# Autodesk Inventor assembly: ELEV_000_FULLASMBLY
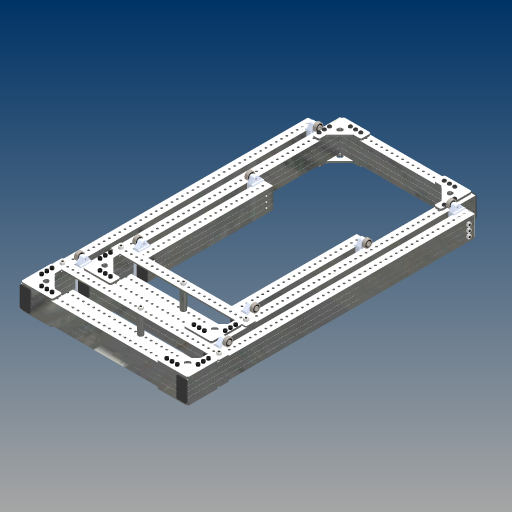
[picture p0: Inventor's stored thumbnail of the model, 512x512]
Saved by Autodesk Inventor 2024.3 (Build 283343000, 343)
## iProperties
Created: 2024-11-25
Part Number: ELEV_000_FULLASMBLY
Document SubType Name: Assembly
Designer: Kenji
Mass: 3407.89 g
Surface Area: 12378 cm^2
Volume: 1206.36 cm^3
Density: 2.82493 g/cm^3
Author: Kenji
## Documents named in this file (30)
- C:\Users\Kenji\Documents\GitHub\1622-2024-Casino-Clash-CAD-A-Thon\Elevator\ELEV_000_FULLASMBLY.iam
- C:\Users\Kenji\Documents\GitHub\1622-2024-Casino-Clash-CAD-A-Thon\Elevator\ELEV_001_BAR1(27.500 in).ipt
- C:\Users\Kenji\Documents\GitHub\1622-2024-Casino-Clash-CAD-A-Thon\Elevator\ELEV_002_BAR2(14.000 in).ipt
- C:\Users\Kenji\Documents\GitHub\1622-2024-Casino-Clash-CAD-A-Thon\Elevator\ELEV_003_BAR3(25.000 in).ipt
- C:\Users\Kenji\Documents\GitHub\1622-2024-Casino-Clash-CAD-A-Thon\COTS Library\Motion\BearingBlocks\ElevatorBlocks\WCP-0897_InlineBearingBlock.iam
- C:\Users\Kenji\Documents\GitHub\1622-2024-Casino-Clash-CAD-A-Thon\Elevator\ELEV_004_BAR4(12.000 in).ipt
- C:\Users\Kenji\Documents\GitHub\1622-2024-Casino-Clash-CAD-A-Thon\Elevator\ELEV_005_SUPBRK1.ipt
- C:\Users\Kenji\Documents\GitHub\1622-2024-Casino-Clash-CAD-A-Thon\COTS Library\Fasteners\Nuts\COTS_90633A411_Low-Strength Steel Thin Nylon-Insert Locknut_10-32.ipt
- C:\Users\Kenji\Documents\GitHub\1622-2024-Casino-Clash-CAD-A-Thon\Elevator\ELEV_006_SUPBRK1_THRD.ipt
- C:\Users\Kenji\Documents\GitHub\1622-2024-Casino-Clash-CAD-A-Thon\COTS Library\Fasteners\Bolts\Socket-Head\10-32\COTS_90044A121_Black-Oxide Alloy Steel Socket Head Screw_10-32_2.5in.ipt
- C:\Users\Kenji\Documents\GitHub\1622-2024-Casino-Clash-CAD-A-Thon\COTS Library\Fasteners\Bolts\Socket-Head\10-32\COTS_90044A202_Black-Oxide Alloy Steel Socket Head Screw_1-.375.ipt
- C:\Users\Kenji\Documents\GitHub\1622-2024-Casino-Clash-CAD-A-Thon\COTS Library\Fasteners\Bolts\Socket-Head\10-32\COTS_91251A342_Black-Oxide Alloy Steel Socket Head Screw_.5in.ipt
- C:\Users\Kenji\Documents\GitHub\1622-2024-Casino-Clash-CAD-A-Thon\Elevator\ELEV_007_SUPBRK2.ipt
- C:\Users\Kenji\Documents\GitHub\1622-2024-Casino-Clash-CAD-A-Thon\COTS Library\Fasteners\Bolts\Socket-Head\10-32\COTS_91251A359_Black-Oxide Alloy Steel Socket Head Screw_10-32_2_3-4in.ipt
- C:\Users\Kenji\Documents\GitHub\1622-2024-Casino-Clash-CAD-A-Thon\COTS Library\Fasteners\Nuts\COTS_90631A411_Low-Strength Steel Nylon-Insert Locknut_10-32.ipt
- C:\Users\Kenji\Documents\GitHub\1622-2024-Casino-Clash-CAD-A-Thon\Elevator\ELEV_008_SUPBRK3.ipt
- C:\Users\Kenji\Documents\GitHub\1622-2024-Casino-Clash-CAD-A-Thon\Elevator\ELEV_010_BOLTCOVER2.ipt
- C:\Users\Kenji\Documents\GitHub\1622-2024-Casino-Clash-CAD-A-Thon\Elevator\ELEV_011_EXTRUENDCAP.ipt
- C:\Users\Kenji\Documents\GitHub\1622-2024-Casino-Clash-CAD-A-Thon\Elevator\ELEV_012_SUPBRK2_THRD.ipt
- C:\Users\Kenji\Documents\GitHub\1622-2024-Casino-Clash-CAD-A-Thon\Elevator\ELEV_013_BAR5(12.000 in).ipt
- C:\Users\Kenji\Documents\GitHub\1622-2024-Casino-Clash-CAD-A-Thon\Elevator\ELEV_015_CRSHBLCK1.ipt
- C:\Users\Kenji\Documents\GitHub\1622-2024-Casino-Clash-CAD-A-Thon\Elevator\ELEV_016_SUPBAR1.ipt
- C:\Users\Kenji\Documents\GitHub\1622-2024-Casino-Clash-CAD-A-Thon\Elevator\ELEV_017_SPACER1.ipt
- C:\Users\Kenji\Documents\GitHub\1622-2024-Casino-Clash-CAD-A-Thon\Elevator\ELEV_018_SUPBAR2.ipt
- C:\Users\Kenji\Documents\GitHub\1622-2024-Casino-Clash-CAD-A-Thon\Elevator\ELEV_000_FULLASMBLY\AIP\FEA\ew6g7bhkw.fins
- C:\Users\Kenji\Documents\GitHub\1622-2024-Casino-Clash-CAD-A-Thon\Elevator\ELEV_000_FULLASMBLY\AIP\FEA\ew6g7bhkw.fsat
- C:\Users\Kenji\Documents\GitHub\1622-2024-Casino-Clash-CAD-A-Thon\Elevator\ELEV_000_FULLASMBLY\AIP\FEA\ew6g7bhkw.ftes
- C:\Users\Kenji\Documents\GitHub\1622-2024-Casino-Clash-CAD-A-Thon\Elevator\ELEV_000_FULLASMBLY\AIP\FEA\ew6g7bhkw.fwiz
- C:\Users\Kenji\Documents\GitHub\1622-2024-Casino-Clash-CAD-A-Thon\Elevator\ELEV_000_FULLASMBLY\AIP\FEA\ew6g7biao.fmsh
- C:\Users\Kenji\Documents\GitHub\1622-2024-Casino-Clash-CAD-A-Thon\Elevator\ELEV_000_FULLASMBLY\AIP\FEA\ew6g7bibk.fres
## Components (192 placed, 23 different names)
1. ELEV_001_BAR1(27.500 in):1 — Flush:1, Flush:2, Mate:1, Mate:2, Flush:7, Tangent:2, Mate:10, Flush:11, Mate:11, Mate:78, Mate:133, Mate:136, Mate:137, Mate:201, Mate:202, Mate:203, Mate:284, Mate:285, Mate:286, Mate:290, Mate:293
2. ELEV_001_BAR1(27.500 in):2 — Flush:1, Flush:2, Mate:1, Flush:3, Flush:4, Mate:3, Angle:1, Mate:4, Flush:8, Angle:2, Mate:74, Mate:128, Mate:131, Mate:198, Mate:199, Mate:200, Mate:287, Mate:288, Mate:289, Mate:291, Mate:292, Mate:294, Mate:295
3. ELEV_002_BAR2(14.000 in):1 — Flush:3, Flush:4, Mate:2, Mate:127, Flush:24, Mate:132, Mate:134, Mate:135
4. ELEV_003_BAR3(25.000 in):1 — Flush:5, Flush:6, Flush:7, Mate:8, Flush:10, Mate:9, Mate:82, Mate:186, Mate:187, Mate:188, Mate:211, Mate:228, Tangent:3, Tangent:4, Angle:5, Angle:6, Mate:265, Mate:266, Mate:267, Mate:312, Mate:313, Mate:316
5. ELEV_003_BAR3(25.000 in):2 — Flush:5, Flush:6, Tangent:1, Angle:2, Mate:5, Angle:3, Mate:6, Flush:9, Mate:12, Flush:12, Flush:13, Mate:13, Flush:14, Mate:14, Mate:16, Mate:62, Mate:86, Mate:189, Mate:190, Mate:191, Mate:192, Mate:193, Mate:194, Mate:207, Mate:208, Tangent:5, Flush:33
6. WCP-0897_InlineBearingBlock:1 [sub-assembly] — Mate:5, Angle:3, Mate:6, Flush:9, Mate:83, Mate:84
7. WCP-0897_InlineBearingBlock:2 [sub-assembly] — Mate:3, Angle:1, Mate:4, Tangent:1, Flush:8, Mate:71, Mate:72
8. WCP-0897_InlineBearingBlock:3 [sub-assembly] — Mate:8, Flush:10, Mate:9, Tangent:2, Mate:79, Mate:80
9. WCP-0897_InlineBearingBlock:4 [sub-assembly] — Mate:10, Flush:11, Mate:11, Mate:75, Mate:76
10. ELEV_004_BAR4(12.000 in):1 — Mate:12, Flush:12, Flush:13, Mate:17, Mate:18, Mate:19, Angle:4, Mate:20, Mate:42, Mate:45, Mate:60, Flush:15, Mate:61, Angle:8
11. ELEV_004_BAR4(12.000 in):2 — Mate:13, Flush:14, Mate:14, Flush:26, Flush:27, Mate:214, Mate:227, Flush:28, Angle:7
12. ELEV_005_SUPBRK1:1 — Mate:16, Mate:17, Mate:18, Mate:67, Mate:68, Mate:69, Mate:70
13. ELEV_005_SUPBRK1:2 — Mate:19, Angle:4, Mate:20, Mate:63, Mate:64, Mate:65, Mate:66
14. ELEV_006_SUPBRK1_THRD:1 — Mate:42, Mate:61, Mate:62, Mate:247, Mate:248
15. ELEV_006_SUPBRK1_THRD:2 — Mate:45, Mate:60, Flush:15, Mate:241, Mate:242, Mate:243, Mate:244
16. ELEV_008_SUPBRK3:1 — Mate:127, Flush:24, Mate:128, Mate:129, Mate:130, Mate:138, Mate:139, Mate:144, Mate:145
17. ELEV_008_SUPBRK3:2 — Mate:129, Mate:130, Mate:131, Mate:148, Mate:149
18. ELEV_008_SUPBRK3:3 — Mate:132, Mate:133, Mate:134, Mate:151, Mate:153
19. ELEV_008_SUPBRK3:4 — Mate:135, Mate:136, Mate:137, Mate:140, Mate:141, Mate:142, Mate:143
20. ELEV_011_EXTRUENDCAP:1 — Mate:189, Mate:190, Mate:191
21. ELEV_011_EXTRUENDCAP:3 — Mate:186, Mate:187, Mate:188, Mate:339
22. ELEV_011_EXTRUENDCAP:5 — Mate:198, Mate:199, Mate:200
23. ELEV_011_EXTRUENDCAP:6 — Mate:201, Mate:202, Mate:203
24. ELEV_011_EXTRUENDCAP:7 — Mate:192, Mate:193, Mate:194
25. ELEV_007_SUPBRK2:1 — Flush:26, Mate:227, Mate:228, Mate:229, Mate:230, Mate:231, Mate:232, Mate:233
26. ELEV_007_SUPBRK2:2 — Flush:27, Mate:207, Mate:208, Mate:212, Mate:213, Mate:217, Mate:218, Mate:219, Mate:220
27. ELEV_012_SUPBRK2_THRD:1 — Mate:211, Mate:229, Flush:28, Mate:239, Mate:240
28. ELEV_012_SUPBRK2_THRD:2 — Mate:212, Mate:213, Mate:214, Mate:235, Mate:332
29. ELEV_013_BAR5(12.000 in):1 — Mate:257, Flush:29, Mate:258, Mate:259, Flush:30, Mate:260, Angle:5, Angle:6, Flush:34, Mate:277, Mate:283, Mate:333, Mate:334, Mate:335
30. ELEV_013_BAR5(12.000 in):2 — Mate:261, Flush:31, Mate:262, Mate:263, Flush:32, Mate:264, Angle:7, Flush:33, Flush:34, Mate:279, Mate:281, Mate:336, Mate:337, Mate:338
31. WCP-0897_InlineBearingBlock:5 [sub-assembly] — Mate:257, Flush:29, Mate:258, Tangent:3, Tangent:4, Mate:270, Mate:271
32. WCP-0897_InlineBearingBlock:6 [sub-assembly] — Mate:259, Flush:30, Mate:260, Mate:274, Mate:275
33. WCP-0897_InlineBearingBlock:7 [sub-assembly] — Mate:261, Flush:31, Mate:262, Tangent:5, Mate:272, Mate:273
34. WCP-0897_InlineBearingBlock:8 [sub-assembly] — Mate:263, Flush:32, Mate:264, Mate:268, Mate:269
35. ELEV_011_EXTRUENDCAP:8 — Mate:265, Mate:266, Mate:267
36. ELEV_015_CRSHBLCK1:1 — Mate:284, Mate:285, Mate:286
37. ELEV_015_CRSHBLCK1:2 — Mate:287, Mate:288, Mate:289
38. ELEV_016_SUPBAR1:1 — Mate:290, Mate:291, Mate:292, Mate:301, Mate:303, Mate:305, Mate:310
39. ELEV_016_SUPBAR1:2 — Mate:293, Mate:294, Mate:295, Mate:296, Mate:297, Mate:298, Mate:299, Mate:304, Mate:306, Mate:307, Mate:308, Mate:339
40. COTS_90044A121_Black-Oxide Alloy Steel Socket Head Screw_10-32_2.5in:27 — Mate:296, Mate:297, Mate:302
41. COTS_90044A121_Black-Oxide Alloy Steel Socket Head Screw_10-32_2.5in:28 — Mate:298, Mate:299, Mate:300
42. COTS_90631A411_Low-Strength Steel Nylon-Insert Locknut_10-32:25 — Mate:300, Mate:301
43. COTS_90631A411_Low-Strength Steel Nylon-Insert Locknut_10-32:26 — Mate:302, Mate:303
44. ELEV_017_SPACER1:1 — Mate:304, Mate:305, Mate:306
45. COTS_90044A121_Black-Oxide Alloy Steel Socket Head Screw_10-32_2.5in:29 — Mate:307, Mate:308, Mate:309
46. COTS_90631A411_Low-Strength Steel Nylon-Insert Locknut_10-32:27 — Mate:309, Mate:310
47. ELEV_018_SUPBAR2:1 — Mate:312, Mate:313, Angle:8, Mate:314, Mate:315, Mate:317, Mate:318, Mate:319, Mate:320, Mate:325, Mate:326, Mate:327, Mate:328, Mate:340
48. ELEV_018_SUPBAR2:2 — Mate:314, Mate:315, Mate:316, Mate:323, Mate:324, Mate:330
49. COTS_90044A121_Black-Oxide Alloy Steel Socket Head Screw_10-32_2.5in:30 — Mate:318, Mate:319, Mate:321
50. COTS_90044A121_Black-Oxide Alloy Steel Socket Head Screw_10-32_2.5in:31 — Mate:317, Mate:320, Mate:322
51. COTS_90044A121_Black-Oxide Alloy Steel Socket Head Screw_10-32_2.5in:32 — Mate:327, Mate:328, Mate:329
52. COTS_90631A411_Low-Strength Steel Nylon-Insert Locknut_10-32:28 — Mate:322, Mate:323
53. COTS_90631A411_Low-Strength Steel Nylon-Insert Locknut_10-32:29 — Mate:321, Mate:324
54. ELEV_017_SPACER1:2 — Mate:325, Mate:326
55. COTS_90631A411_Low-Strength Steel Nylon-Insert Locknut_10-32:30 — Mate:329, Mate:330
56. ELEV_011_EXTRUENDCAP:9 — Mate:333, Mate:334, Mate:335, Mate:340
57. ELEV_011_EXTRUENDCAP:10 — Mate:336, Mate:337, Mate:338
58. COTS_90044A121_Black-Oxide Alloy Steel Socket Head Screw_10-32_2.5in:1 — Mate:63, Mate:64
59. COTS_90044A121_Black-Oxide Alloy Steel Socket Head Screw_10-32_2.5in:5
60. COTS_90044A121_Black-Oxide Alloy Steel Socket Head Screw_10-32_2.5in:6
61. COTS_90044A121_Black-Oxide Alloy Steel Socket Head Screw_10-32_2.5in:4 — Mate:65, Mate:66
62. COTS_90044A121_Black-Oxide Alloy Steel Socket Head Screw_10-32_2.5in:7
63. COTS_90044A121_Black-Oxide Alloy Steel Socket Head Screw_10-32_2.5in:8
64. COTS_90044A121_Black-Oxide Alloy Steel Socket Head Screw_10-32_2.5in:2 — Mate:67, Mate:69, Mate:245
65. COTS_90044A121_Black-Oxide Alloy Steel Socket Head Screw_10-32_2.5in:11
66. COTS_90044A121_Black-Oxide Alloy Steel Socket Head Screw_10-32_2.5in:12
67. COTS_90044A202_Black-Oxide Alloy Steel Socket Head Screw_1-.375:1 — Mate:71, Mate:72, Mate:73
68. COTS_90633A411_Low-Strength Steel Thin Nylon-Insert Locknut_10-32:1 — Mate:73, Mate:74
69. COTS_90044A202_Black-Oxide Alloy Steel Socket Head Screw_1-.375:2
70. COTS_90633A411_Low-Strength Steel Thin Nylon-Insert Locknut_10-32:2
71. COTS_90044A202_Black-Oxide Alloy Steel Socket Head Screw_1-.375:3
72. COTS_90633A411_Low-Strength Steel Thin Nylon-Insert Locknut_10-32:3
73. COTS_90633A411_Low-Strength Steel Thin Nylon-Insert Locknut_10-32:4 — Mate:77, Mate:78
74. COTS_90044A202_Black-Oxide Alloy Steel Socket Head Screw_1-.375:4 — Mate:75, Mate:76, Mate:77
75. COTS_90633A411_Low-Strength Steel Thin Nylon-Insert Locknut_10-32:5
76. COTS_90044A202_Black-Oxide Alloy Steel Socket Head Screw_1-.375:5
77. COTS_90633A411_Low-Strength Steel Thin Nylon-Insert Locknut_10-32:6
78. COTS_90044A202_Black-Oxide Alloy Steel Socket Head Screw_1-.375:6
79. COTS_91251A342_Black-Oxide Alloy Steel Socket Head Screw_.5in:1 — Mate:79, Mate:80, Mate:81
80. COTS_90633A411_Low-Strength Steel Thin Nylon-Insert Locknut_10-32:7 — Mate:81, Mate:82
81. COTS_91251A342_Black-Oxide Alloy Steel Socket Head Screw_.5in:2
82. COTS_90633A411_Low-Strength Steel Thin Nylon-Insert Locknut_10-32:8
83. COTS_91251A342_Black-Oxide Alloy Steel Socket Head Screw_.5in:3
84. COTS_90633A411_Low-Strength Steel Thin Nylon-Insert Locknut_10-32:9
85. COTS_90633A411_Low-Strength Steel Thin Nylon-Insert Locknut_10-32:10 — Mate:85, Mate:86
86. COTS_91251A342_Black-Oxide Alloy Steel Socket Head Screw_.5in:4 — Mate:83, Mate:84, Mate:85
87. COTS_90633A411_Low-Strength Steel Thin Nylon-Insert Locknut_10-32:11
88. COTS_91251A342_Black-Oxide Alloy Steel Socket Head Screw_.5in:5
89. COTS_90633A411_Low-Strength Steel Thin Nylon-Insert Locknut_10-32:12
90. COTS_91251A342_Black-Oxide Alloy Steel Socket Head Screw_.5in:6
91. COTS_90631A411_Low-Strength Steel Nylon-Insert Locknut_10-32:14 — Mate:152, Mate:153, Mate:255
92. COTS_91251A359_Black-Oxide Alloy Steel Socket Head Screw_10-32_2_3-4in:14 — Mate:140, Mate:143, Mate:152, Mate:249
93. COTS_90631A411_Low-Strength Steel Nylon-Insert Locknut_10-32:17
94. COTS_91251A359_Black-Oxide Alloy Steel Socket Head Screw_10-32_2_3-4in:17
95. COTS_90631A411_Low-Strength Steel Nylon-Insert Locknut_10-32:18
96. COTS_91251A359_Black-Oxide Alloy Steel Socket Head Screw_10-32_2_3-4in:18
97. COTS_91251A359_Black-Oxide Alloy Steel Socket Head Screw_10-32_2_3-4in:13 — Mate:141, Mate:142, Mate:150, Mate:250
98. COTS_90631A411_Low-Strength Steel Nylon-Insert Locknut_10-32:15 — Mate:150, Mate:151, Mate:256
99. COTS_91251A359_Black-Oxide Alloy Steel Socket Head Screw_10-32_2_3-4in:19
100. COTS_90631A411_Low-Strength Steel Nylon-Insert Locknut_10-32:19
101. COTS_91251A359_Black-Oxide Alloy Steel Socket Head Screw_10-32_2_3-4in:20
102. COTS_90631A411_Low-Strength Steel Nylon-Insert Locknut_10-32:20
103. COTS_91251A359_Black-Oxide Alloy Steel Socket Head Screw_10-32_2_3-4in:15 — Mate:139, Mate:145, Mate:147
104. COTS_90631A411_Low-Strength Steel Nylon-Insert Locknut_10-32:13 — Mate:147, Mate:149
105. COTS_91251A359_Black-Oxide Alloy Steel Socket Head Screw_10-32_2_3-4in:21
106. COTS_90631A411_Low-Strength Steel Nylon-Insert Locknut_10-32:21
107. COTS_91251A359_Black-Oxide Alloy Steel Socket Head Screw_10-32_2_3-4in:22 — Mate:251
108. COTS_90631A411_Low-Strength Steel Nylon-Insert Locknut_10-32:22 — Mate:254
109. COTS_90631A411_Low-Strength Steel Nylon-Insert Locknut_10-32:16 — Mate:146, Mate:148, Mate:253
110. COTS_91251A359_Black-Oxide Alloy Steel Socket Head Screw_10-32_2_3-4in:16 — Mate:138, Mate:144, Mate:146, Mate:252
111. COTS_90631A411_Low-Strength Steel Nylon-Insert Locknut_10-32:23
112. COTS_91251A359_Black-Oxide Alloy Steel Socket Head Screw_10-32_2_3-4in:23
113. COTS_90631A411_Low-Strength Steel Nylon-Insert Locknut_10-32:24
114. COTS_91251A359_Black-Oxide Alloy Steel Socket Head Screw_10-32_2_3-4in:24
115. COTS_90044A121_Black-Oxide Alloy Steel Socket Head Screw_10-32_2.5in:15 — Mate:230, Mate:233, Mate:237
116. ELEV_010_BOLTCOVER2:28 — Mate:237, Mate:240
117. COTS_90044A121_Black-Oxide Alloy Steel Socket Head Screw_10-32_2.5in:17
118. ELEV_010_BOLTCOVER2:29
119. COTS_90044A121_Black-Oxide Alloy Steel Socket Head Screw_10-32_2.5in:18
120. ELEV_010_BOLTCOVER2:30
121. ELEV_010_BOLTCOVER2:26 — Mate:238, Mate:239
122. COTS_90044A121_Black-Oxide Alloy Steel Socket Head Screw_10-32_2.5in:14 — Mate:231, Mate:232, Mate:238
123. ELEV_010_BOLTCOVER2:31
124. COTS_90044A121_Black-Oxide Alloy Steel Socket Head Screw_10-32_2.5in:19
125. ELEV_010_BOLTCOVER2:32
126. COTS_90044A121_Black-Oxide Alloy Steel Socket Head Screw_10-32_2.5in:20
127. COTS_90044A121_Black-Oxide Alloy Steel Socket Head Screw_10-32_2.5in:13 — Mate:217, Mate:220, Mate:234
128. ELEV_010_BOLTCOVER2:25 — Mate:234, Mate:235
129. COTS_90044A121_Black-Oxide Alloy Steel Socket Head Screw_10-32_2.5in:21
130. ELEV_010_BOLTCOVER2:33
131. COTS_90044A121_Black-Oxide Alloy Steel Socket Head Screw_10-32_2.5in:22
132. ELEV_010_BOLTCOVER2:34
133. COTS_90044A121_Black-Oxide Alloy Steel Socket Head Screw_10-32_2.5in:16 — Mate:218, Mate:219, Mate:236, Mate:331
134. ELEV_010_BOLTCOVER2:27 — Mate:236
135. COTS_90044A121_Black-Oxide Alloy Steel Socket Head Screw_10-32_2.5in:23
136. ELEV_010_BOLTCOVER2:35
137. COTS_90044A121_Black-Oxide Alloy Steel Socket Head Screw_10-32_2.5in:24
138. ELEV_010_BOLTCOVER2:36
139. ELEV_010_BOLTCOVER2:38 — Mate:242, Mate:243
140. ELEV_010_BOLTCOVER2:41
141. ELEV_010_BOLTCOVER2:42
142. ELEV_010_BOLTCOVER2:37 — Mate:241, Mate:244
143. ELEV_010_BOLTCOVER2:43
144. ELEV_010_BOLTCOVER2:44
145. ELEV_010_BOLTCOVER2:40 — Mate:245, Mate:248
146. ELEV_010_BOLTCOVER2:45
147. ELEV_010_BOLTCOVER2:46
148. ELEV_010_BOLTCOVER2:39 — Mate:246, Mate:247
149. COTS_90044A121_Black-Oxide Alloy Steel Socket Head Screw_10-32_2.5in:3 — Mate:68, Mate:70, Mate:246
150. ELEV_010_BOLTCOVER2:47
151. COTS_90044A121_Black-Oxide Alloy Steel Socket Head Screw_10-32_2.5in:25
152. ELEV_010_BOLTCOVER2:48
153. COTS_90044A121_Black-Oxide Alloy Steel Socket Head Screw_10-32_2.5in:26
154. ELEV_010_BOLTCOVER2:50 — Mate:250, Mate:256
155. ELEV_010_BOLTCOVER2:53
156. ELEV_010_BOLTCOVER2:54
157. ELEV_010_BOLTCOVER2:49 — Mate:249, Mate:255
158. ELEV_010_BOLTCOVER2:55
159. ELEV_010_BOLTCOVER2:56
160. ELEV_010_BOLTCOVER2:51 — Mate:251, Mate:254
161. ELEV_010_BOLTCOVER2:57
162. ELEV_010_BOLTCOVER2:58
163. ELEV_010_BOLTCOVER2:52 — Mate:252, Mate:253
164. ELEV_010_BOLTCOVER2:59
165. ELEV_010_BOLTCOVER2:60
166. COTS_90633A411_Low-Strength Steel Thin Nylon-Insert Locknut_10-32:16 — Mate:282, Mate:283
167. COTS_91251A342_Black-Oxide Alloy Steel Socket Head Screw_.5in:7 — Mate:274, Mate:275, Mate:282
168. COTS_90633A411_Low-Strength Steel Thin Nylon-Insert Locknut_10-32:17
169. COTS_91251A342_Black-Oxide Alloy Steel Socket Head Screw_.5in:11
170. COTS_90633A411_Low-Strength Steel Thin Nylon-Insert Locknut_10-32:18
171. COTS_91251A342_Black-Oxide Alloy Steel Socket Head Screw_.5in:12
172. COTS_91251A342_Black-Oxide Alloy Steel Socket Head Screw_.5in:10 — Mate:270, Mate:271, Mate:276
173. COTS_90633A411_Low-Strength Steel Thin Nylon-Insert Locknut_10-32:13 — Mate:276, Mate:277
174. COTS_91251A342_Black-Oxide Alloy Steel Socket Head Screw_.5in:13
175. COTS_90633A411_Low-Strength Steel Thin Nylon-Insert Locknut_10-32:19
176. COTS_91251A342_Black-Oxide Alloy Steel Socket Head Screw_.5in:14
177. COTS_90633A411_Low-Strength Steel Thin Nylon-Insert Locknut_10-32:20
178. COTS_90633A411_Low-Strength Steel Thin Nylon-Insert Locknut_10-32:14 — Mate:278, Mate:279
179. COTS_91251A342_Black-Oxide Alloy Steel Socket Head Screw_.5in:9 — Mate:268, Mate:269, Mate:278
180. COTS_90633A411_Low-Strength Steel Thin Nylon-Insert Locknut_10-32:21
181. COTS_91251A342_Black-Oxide Alloy Steel Socket Head Screw_.5in:15
182. COTS_90633A411_Low-Strength Steel Thin Nylon-Insert Locknut_10-32:22
183. COTS_91251A342_Black-Oxide Alloy Steel Socket Head Screw_.5in:16
184. COTS_91251A342_Black-Oxide Alloy Steel Socket Head Screw_.5in:8 — Mate:272, Mate:273, Mate:280
185. COTS_90633A411_Low-Strength Steel Thin Nylon-Insert Locknut_10-32:15 — Mate:280, Mate:281
186. COTS_91251A342_Black-Oxide Alloy Steel Socket Head Screw_.5in:17
187. COTS_90633A411_Low-Strength Steel Thin Nylon-Insert Locknut_10-32:23
188. COTS_91251A342_Black-Oxide Alloy Steel Socket Head Screw_.5in:18
189. COTS_90633A411_Low-Strength Steel Thin Nylon-Insert Locknut_10-32:24
190. ELEV_010_BOLTCOVER2:61 — Mate:331, Mate:332
191. ELEV_010_BOLTCOVER2:62
192. ELEV_010_BOLTCOVER2:63
## Component patterns: (3 elements, first: COTS_90044A121_Black-Oxide Alloy Steel Socket Head Screw_10-32_2.5in:1), (3 elements, first: COTS_90044A121_Black-Oxide Alloy Steel Socket Head Screw_10-32_2.5in:4), (3 elements, first: COTS_90044A121_Black-Oxide Alloy Steel Socket Head Screw_10-32_2.5in:2), (3 elements, first: COTS_90044A202_Black-Oxide Alloy Steel Socket Head Screw_1-.375:1 + COTS_90633A411_Low-Strength Steel Thin Nylon-Insert Locknut_10-32:1), (3 elements, first: COTS_90633A411_Low-Strength Steel Thin Nylon-Insert Locknut_10-32:4 + COTS_90044A202_Black-Oxide Alloy Steel Socket Head Screw_1-.375:4), (3 elements, first: COTS_91251A342_Black-Oxide Alloy Steel Socket Head Screw_.5in:1 + COTS_90633A411_Low-Strength Steel Thin Nylon-Insert Locknut_10-32:7), (3 elements, first: COTS_90633A411_Low-Strength Steel Thin Nylon-Insert Locknut_10-32:10 + COTS_91251A342_Black-Oxide Alloy Steel Socket Head Screw_.5in:4), (3 elements, first: COTS_90631A411_Low-Strength Steel Nylon-Insert Locknut_10-32:14 + COTS_91251A359_Black-Oxide Alloy Steel Socket Head Screw_10-32_2_3-4in:14), (3 elements, first: COTS_91251A359_Black-Oxide Alloy Steel Socket Head Screw_10-32_2_3-4in:13 + COTS_90631A411_Low-Strength Steel Nylon-Insert Locknut_10-32:15), (3 elements, first: COTS_91251A359_Black-Oxide Alloy Steel Socket Head Screw_10-32_2_3-4in:15 + COTS_90631A411_Low-Strength Steel Nylon-Insert Locknut_10-32:13), (3 elements, first: COTS_90631A411_Low-Strength Steel Nylon-Insert Locknut_10-32:16 + COTS_91251A359_Black-Oxide Alloy Steel Socket Head Screw_10-32_2_3-4in:16), (3 elements, first: COTS_90044A121_Black-Oxide Alloy Steel Socket Head Screw_10-32_2.5in:15 + ELEV_010_BOLTCOVER2:28), (3 elements, first: ELEV_010_BOLTCOVER2:26 + COTS_90044A121_Black-Oxide Alloy Steel Socket Head Screw_10-32_2.5in:14), (3 elements, first: COTS_90044A121_Black-Oxide Alloy Steel Socket Head Screw_10-32_2.5in:13 + ELEV_010_BOLTCOVER2:25), (3 elements, first: COTS_90044A121_Black-Oxide Alloy Steel Socket Head Screw_10-32_2.5in:16 + ELEV_010_BOLTCOVER2:27), (3 elements, first: ELEV_010_BOLTCOVER2:38), (3 elements, first: ELEV_010_BOLTCOVER2:37), (3 elements, first: ELEV_010_BOLTCOVER2:40), (3 elements, first: ELEV_010_BOLTCOVER2:39 + COTS_90044A121_Black-Oxide Alloy Steel Socket Head Screw_10-32_2.5in:3), (3 elements, first: ELEV_010_BOLTCOVER2:50), (3 elements, first: ELEV_010_BOLTCOVER2:49), (3 elements, first: ELEV_010_BOLTCOVER2:51), (3 elements, first: ELEV_010_BOLTCOVER2:52), (3 elements, first: COTS_90633A411_Low-Strength Steel Thin Nylon-Insert Locknut_10-32:16 + COTS_91251A342_Black-Oxide Alloy Steel Socket Head Screw_.5in:7), (3 elements, first: COTS_91251A342_Black-Oxide Alloy Steel Socket Head Screw_.5in:10 + COTS_90633A411_Low-Strength Steel Thin Nylon-Insert Locknut_10-32:13), (3 elements, first: COTS_90633A411_Low-Strength Steel Thin Nylon-Insert Locknut_10-32:14 + COTS_91251A342_Black-Oxide Alloy Steel Socket Head Screw_.5in:9), (3 elements, first: COTS_91251A342_Black-Oxide Alloy Steel Socket Head Screw_.5in:8 + COTS_90633A411_Low-Strength Steel Thin Nylon-Insert Locknut_10-32:15), (3 elements, first: ELEV_010_BOLTCOVER2:61)
## Relationships (250: Mate 212, Flush 25, Angle 8, Tangent 5)
- Flush:1: ELEV_001_BAR1(27.500 in):1 ↔ ELEV_001_BAR1(27.500 in):2
- Flush:2: ELEV_001_BAR1(27.500 in):1 ↔ ELEV_001_BAR1(27.500 in):2
- Mate:1 (355.6 mm): ELEV_001_BAR1(27.500 in):1 ↔ ELEV_001_BAR1(27.500 in):2
- Flush:3: ELEV_001_BAR1(27.500 in):2 ↔ ELEV_002_BAR2(14.000 in):1
- Flush:4: ELEV_001_BAR1(27.500 in):2 ↔ ELEV_002_BAR2(14.000 in):1
- Mate:2: ELEV_001_BAR1(27.500 in):1 ↔ ELEV_002_BAR2(14.000 in):1
- Flush:5: ELEV_003_BAR3(25.000 in):1 ↔ ELEV_003_BAR3(25.000 in):2
- Flush:6: ELEV_003_BAR3(25.000 in):1 ↔ ELEV_003_BAR3(25.000 in):2
- Flush:7: ELEV_001_BAR1(27.500 in):1 ↔ ELEV_003_BAR3(25.000 in):1
- Mate:3: ELEV_001_BAR1(27.500 in):2 ↔ WCP-0897_InlineBearingBlock:2
- Angle:1 (0 deg): ELEV_001_BAR1(27.500 in):2 ↔ WCP-0897_InlineBearingBlock:2
- Mate:4: ELEV_001_BAR1(27.500 in):2 ↔ WCP-0897_InlineBearingBlock:2
- Tangent:1: ELEV_003_BAR3(25.000 in):2 ↔ WCP-0897_InlineBearingBlock:2
- Flush:8: ELEV_001_BAR1(27.500 in):2 ↔ WCP-0897_InlineBearingBlock:2
- Angle:2 (0 deg): ELEV_001_BAR1(27.500 in):2 ↔ ELEV_003_BAR3(25.000 in):2
- Mate:5: ELEV_003_BAR3(25.000 in):2 ↔ WCP-0897_InlineBearingBlock:1
- Angle:3 (0 deg): ELEV_003_BAR3(25.000 in):2 ↔ WCP-0897_InlineBearingBlock:1
- Mate:6: ELEV_003_BAR3(25.000 in):2 ↔ WCP-0897_InlineBearingBlock:1
- Flush:9: ELEV_003_BAR3(25.000 in):2 ↔ WCP-0897_InlineBearingBlock:1
- Mate:8: ELEV_003_BAR3(25.000 in):1 ↔ WCP-0897_InlineBearingBlock:3
- Flush:10: ELEV_003_BAR3(25.000 in):1 ↔ WCP-0897_InlineBearingBlock:3
- Mate:9: ELEV_003_BAR3(25.000 in):1 ↔ WCP-0897_InlineBearingBlock:3
- Tangent:2: ELEV_001_BAR1(27.500 in):1 ↔ WCP-0897_InlineBearingBlock:3
- Mate:10: ELEV_001_BAR1(27.500 in):1 ↔ WCP-0897_InlineBearingBlock:4
- Flush:11: ELEV_001_BAR1(27.500 in):1 ↔ WCP-0897_InlineBearingBlock:4
- Mate:11: ELEV_001_BAR1(27.500 in):1 ↔ WCP-0897_InlineBearingBlock:4
- Mate:12: ELEV_003_BAR3(25.000 in):2 ↔ ELEV_004_BAR4(12.000 in):1
- Flush:12: ELEV_003_BAR3(25.000 in):2 ↔ ELEV_004_BAR4(12.000 in):1
- Flush:13: ELEV_003_BAR3(25.000 in):2 ↔ ELEV_004_BAR4(12.000 in):1
- Mate:13: ELEV_003_BAR3(25.000 in):2 ↔ ELEV_004_BAR4(12.000 in):2
- Flush:14: ELEV_003_BAR3(25.000 in):2 ↔ ELEV_004_BAR4(12.000 in):2
- Mate:14: ELEV_003_BAR3(25.000 in):2 ↔ ELEV_004_BAR4(12.000 in):2
- Mate:16: ELEV_003_BAR3(25.000 in):2 ↔ ELEV_005_SUPBRK1:1
- Mate:17: ELEV_004_BAR4(12.000 in):1 ↔ ELEV_005_SUPBRK1:1
- Mate:18: ELEV_004_BAR4(12.000 in):1 ↔ ELEV_005_SUPBRK1:1
- Mate:19: ELEV_004_BAR4(12.000 in):1 ↔ ELEV_005_SUPBRK1:2
- Angle:4 (0 deg): ELEV_004_BAR4(12.000 in):1 ↔ ELEV_005_SUPBRK1:2
- Mate:20: ELEV_004_BAR4(12.000 in):1 ↔ ELEV_005_SUPBRK1:2
- Mate:42: ELEV_004_BAR4(12.000 in):1 ↔ ELEV_006_SUPBRK1_THRD:1
- Mate:45: ELEV_004_BAR4(12.000 in):1 ↔ ELEV_006_SUPBRK1_THRD:2
- Mate:60: ELEV_004_BAR4(12.000 in):1 ↔ ELEV_006_SUPBRK1_THRD:2
- Flush:15: ELEV_004_BAR4(12.000 in):1 ↔ ELEV_006_SUPBRK1_THRD:2
- Mate:61: ELEV_004_BAR4(12.000 in):1 ↔ ELEV_006_SUPBRK1_THRD:1
- Mate:62: ELEV_003_BAR3(25.000 in):2 ↔ ELEV_006_SUPBRK1_THRD:1
- Mate:63: ELEV_005_SUPBRK1:2 ↔ COTS_90044A121_Black-Oxide Alloy Steel Socket Head Screw_10-32_2.5in:1
- Mate:64: ELEV_005_SUPBRK1:2 ↔ COTS_90044A121_Black-Oxide Alloy Steel Socket Head Screw_10-32_2.5in:1
- Mate:65: ELEV_005_SUPBRK1:2 ↔ COTS_90044A121_Black-Oxide Alloy Steel Socket Head Screw_10-32_2.5in:4
- Mate:66: ELEV_005_SUPBRK1:2 ↔ COTS_90044A121_Black-Oxide Alloy Steel Socket Head Screw_10-32_2.5in:4
- Mate:67: ELEV_005_SUPBRK1:1 ↔ COTS_90044A121_Black-Oxide Alloy Steel Socket Head Screw_10-32_2.5in:2
- Mate:68: ELEV_005_SUPBRK1:1 ↔ COTS_90044A121_Black-Oxide Alloy Steel Socket Head Screw_10-32_2.5in:3
- Mate:69: ELEV_005_SUPBRK1:1 ↔ COTS_90044A121_Black-Oxide Alloy Steel Socket Head Screw_10-32_2.5in:2
- Mate:70: ELEV_005_SUPBRK1:1 ↔ COTS_90044A121_Black-Oxide Alloy Steel Socket Head Screw_10-32_2.5in:3
- Mate:71: WCP-0897_InlineBearingBlock:2 ↔ COTS_90044A202_Black-Oxide Alloy Steel Socket Head Screw_1-.375:1
- Mate:72: WCP-0897_InlineBearingBlock:2 ↔ COTS_90044A202_Black-Oxide Alloy Steel Socket Head Screw_1-.375:1
- Mate:73: COTS_90044A202_Black-Oxide Alloy Steel Socket Head Screw_1-.375:1 ↔ COTS_90633A411_Low-Strength Steel Thin Nylon-Insert Locknut_10-32:1
- Mate:74: ELEV_001_BAR1(27.500 in):2 ↔ COTS_90633A411_Low-Strength Steel Thin Nylon-Insert Locknut_10-32:1
- Mate:75: WCP-0897_InlineBearingBlock:4 ↔ COTS_90044A202_Black-Oxide Alloy Steel Socket Head Screw_1-.375:4
- Mate:76: WCP-0897_InlineBearingBlock:4 ↔ COTS_90044A202_Black-Oxide Alloy Steel Socket Head Screw_1-.375:4
- Mate:77: COTS_90633A411_Low-Strength Steel Thin Nylon-Insert Locknut_10-32:4 ↔ COTS_90044A202_Black-Oxide Alloy Steel Socket Head Screw_1-.375:4
- Mate:78: ELEV_001_BAR1(27.500 in):1 ↔ COTS_90633A411_Low-Strength Steel Thin Nylon-Insert Locknut_10-32:4
- Mate:79: WCP-0897_InlineBearingBlock:3 ↔ COTS_91251A342_Black-Oxide Alloy Steel Socket Head Screw_.5in:1
- Mate:80: WCP-0897_InlineBearingBlock:3 ↔ COTS_91251A342_Black-Oxide Alloy Steel Socket Head Screw_.5in:1
- Mate:81: COTS_91251A342_Black-Oxide Alloy Steel Socket Head Screw_.5in:1 ↔ COTS_90633A411_Low-Strength Steel Thin Nylon-Insert Locknut_10-32:7
- Mate:82: ELEV_003_BAR3(25.000 in):1 ↔ COTS_90633A411_Low-Strength Steel Thin Nylon-Insert Locknut_10-32:7
- Mate:83: WCP-0897_InlineBearingBlock:1 ↔ COTS_91251A342_Black-Oxide Alloy Steel Socket Head Screw_.5in:4
- Mate:84: WCP-0897_InlineBearingBlock:1 ↔ COTS_91251A342_Black-Oxide Alloy Steel Socket Head Screw_.5in:4
- Mate:85: COTS_90633A411_Low-Strength Steel Thin Nylon-Insert Locknut_10-32:10 ↔ COTS_91251A342_Black-Oxide Alloy Steel Socket Head Screw_.5in:4
- Mate:86: ELEV_003_BAR3(25.000 in):2 ↔ COTS_90633A411_Low-Strength Steel Thin Nylon-Insert Locknut_10-32:10
- Mate:127: ELEV_002_BAR2(14.000 in):1 ↔ ELEV_008_SUPBRK3:1
- Flush:24: ELEV_002_BAR2(14.000 in):1 ↔ ELEV_008_SUPBRK3:1
- Mate:128: ELEV_001_BAR1(27.500 in):2 ↔ ELEV_008_SUPBRK3:1
- Mate:129: ELEV_008_SUPBRK3:1 ↔ ELEV_008_SUPBRK3:2
- Mate:130: ELEV_008_SUPBRK3:1 ↔ ELEV_008_SUPBRK3:2
- Mate:131: ELEV_001_BAR1(27.500 in):2 ↔ ELEV_008_SUPBRK3:2
- Mate:132: ELEV_002_BAR2(14.000 in):1 ↔ ELEV_008_SUPBRK3:3
- Mate:133: ELEV_001_BAR1(27.500 in):1 ↔ ELEV_008_SUPBRK3:3
- Mate:134: ELEV_002_BAR2(14.000 in):1 ↔ ELEV_008_SUPBRK3:3
- Mate:135: ELEV_002_BAR2(14.000 in):1 ↔ ELEV_008_SUPBRK3:4
- Mate:136: ELEV_001_BAR1(27.500 in):1 ↔ ELEV_008_SUPBRK3:4
- Mate:137: ELEV_001_BAR1(27.500 in):1 ↔ ELEV_008_SUPBRK3:4
- Mate:138: ELEV_008_SUPBRK3:1 ↔ COTS_91251A359_Black-Oxide Alloy Steel Socket Head Screw_10-32_2_3-4in:16
- Mate:139: ELEV_008_SUPBRK3:1 ↔ COTS_91251A359_Black-Oxide Alloy Steel Socket Head Screw_10-32_2_3-4in:15
- Mate:140: ELEV_008_SUPBRK3:4 ↔ COTS_91251A359_Black-Oxide Alloy Steel Socket Head Screw_10-32_2_3-4in:14
- Mate:141: ELEV_008_SUPBRK3:4 ↔ COTS_91251A359_Black-Oxide Alloy Steel Socket Head Screw_10-32_2_3-4in:13
- Mate:142: ELEV_008_SUPBRK3:4 ↔ COTS_91251A359_Black-Oxide Alloy Steel Socket Head Screw_10-32_2_3-4in:13
- Mate:143: ELEV_008_SUPBRK3:4 ↔ COTS_91251A359_Black-Oxide Alloy Steel Socket Head Screw_10-32_2_3-4in:14
- Mate:144: ELEV_008_SUPBRK3:1 ↔ COTS_91251A359_Black-Oxide Alloy Steel Socket Head Screw_10-32_2_3-4in:16
- Mate:145: ELEV_008_SUPBRK3:1 ↔ COTS_91251A359_Black-Oxide Alloy Steel Socket Head Screw_10-32_2_3-4in:15
- Mate:146: COTS_90631A411_Low-Strength Steel Nylon-Insert Locknut_10-32:16 ↔ COTS_91251A359_Black-Oxide Alloy Steel Socket Head Screw_10-32_2_3-4in:16
- Mate:147: COTS_91251A359_Black-Oxide Alloy Steel Socket Head Screw_10-32_2_3-4in:15 ↔ COTS_90631A411_Low-Strength Steel Nylon-Insert Locknut_10-32:13
- Mate:148: ELEV_008_SUPBRK3:2 ↔ COTS_90631A411_Low-Strength Steel Nylon-Insert Locknut_10-32:16
- Mate:149: ELEV_008_SUPBRK3:2 ↔ COTS_90631A411_Low-Strength Steel Nylon-Insert Locknut_10-32:13
- Mate:150: COTS_91251A359_Black-Oxide Alloy Steel Socket Head Screw_10-32_2_3-4in:13 ↔ COTS_90631A411_Low-Strength Steel Nylon-Insert Locknut_10-32:15
- Mate:151: ELEV_008_SUPBRK3:3 ↔ COTS_90631A411_Low-Strength Steel Nylon-Insert Locknut_10-32:15
- Mate:152: COTS_90631A411_Low-Strength Steel Nylon-Insert Locknut_10-32:14 ↔ COTS_91251A359_Black-Oxide Alloy Steel Socket Head Screw_10-32_2_3-4in:14
- Mate:153: ELEV_008_SUPBRK3:3 ↔ COTS_90631A411_Low-Strength Steel Nylon-Insert Locknut_10-32:14
- Mate:186: ELEV_003_BAR3(25.000 in):1 ↔ ELEV_011_EXTRUENDCAP:3
- Mate:187: ELEV_003_BAR3(25.000 in):1 ↔ ELEV_011_EXTRUENDCAP:3
- Mate:188: ELEV_003_BAR3(25.000 in):1 ↔ ELEV_011_EXTRUENDCAP:3
- Mate:189: ELEV_003_BAR3(25.000 in):2 ↔ ELEV_011_EXTRUENDCAP:1
- Mate:190: ELEV_003_BAR3(25.000 in):2 ↔ ELEV_011_EXTRUENDCAP:1
- Mate:191: ELEV_003_BAR3(25.000 in):2 ↔ ELEV_011_EXTRUENDCAP:1
- Mate:192: ELEV_003_BAR3(25.000 in):2 ↔ ELEV_011_EXTRUENDCAP:7
- Mate:193: ELEV_003_BAR3(25.000 in):2 ↔ ELEV_011_EXTRUENDCAP:7
- Mate:194: ELEV_003_BAR3(25.000 in):2 ↔ ELEV_011_EXTRUENDCAP:7
- Mate:198: ELEV_001_BAR1(27.500 in):2 ↔ ELEV_011_EXTRUENDCAP:5
- Mate:199: ELEV_001_BAR1(27.500 in):2 ↔ ELEV_011_EXTRUENDCAP:5
- Mate:200: ELEV_001_BAR1(27.500 in):2 ↔ ELEV_011_EXTRUENDCAP:5
- Mate:201: ELEV_001_BAR1(27.500 in):1 ↔ ELEV_011_EXTRUENDCAP:6
- Mate:202: ELEV_001_BAR1(27.500 in):1 ↔ ELEV_011_EXTRUENDCAP:6
- Mate:203: ELEV_001_BAR1(27.500 in):1 ↔ ELEV_011_EXTRUENDCAP:6
- Flush:26: ELEV_004_BAR4(12.000 in):2 ↔ ELEV_007_SUPBRK2:1
- Flush:27: ELEV_004_BAR4(12.000 in):2 ↔ ELEV_007_SUPBRK2:2
- Mate:207: ELEV_003_BAR3(25.000 in):2 ↔ ELEV_007_SUPBRK2:2
- Mate:208: ELEV_003_BAR3(25.000 in):2 ↔ ELEV_007_SUPBRK2:2
- Mate:211: ELEV_003_BAR3(25.000 in):1 ↔ ELEV_012_SUPBRK2_THRD:1
- Mate:212: ELEV_007_SUPBRK2:2 ↔ ELEV_012_SUPBRK2_THRD:2
- Mate:213: ELEV_007_SUPBRK2:2 ↔ ELEV_012_SUPBRK2_THRD:2
- Mate:214: ELEV_004_BAR4(12.000 in):2 ↔ ELEV_012_SUPBRK2_THRD:2
- Mate:217: ELEV_007_SUPBRK2:2 ↔ COTS_90044A121_Black-Oxide Alloy Steel Socket Head Screw_10-32_2.5in:13
- Mate:218: ELEV_007_SUPBRK2:2 ↔ COTS_90044A121_Black-Oxide Alloy Steel Socket Head Screw_10-32_2.5in:16
- Mate:219: ELEV_007_SUPBRK2:2 ↔ COTS_90044A121_Black-Oxide Alloy Steel Socket Head Screw_10-32_2.5in:16
- Mate:220: ELEV_007_SUPBRK2:2 ↔ COTS_90044A121_Black-Oxide Alloy Steel Socket Head Screw_10-32_2.5in:13
- Mate:227: ELEV_004_BAR4(12.000 in):2 ↔ ELEV_007_SUPBRK2:1
- Mate:228: ELEV_003_BAR3(25.000 in):1 ↔ ELEV_007_SUPBRK2:1
- Mate:229: ELEV_007_SUPBRK2:1 ↔ ELEV_012_SUPBRK2_THRD:1
- Flush:28: ELEV_004_BAR4(12.000 in):2 ↔ ELEV_012_SUPBRK2_THRD:1
- Mate:230: ELEV_007_SUPBRK2:1 ↔ COTS_90044A121_Black-Oxide Alloy Steel Socket Head Screw_10-32_2.5in:15
- Mate:231: ELEV_007_SUPBRK2:1 ↔ COTS_90044A121_Black-Oxide Alloy Steel Socket Head Screw_10-32_2.5in:14
- Mate:232: ELEV_007_SUPBRK2:1 ↔ COTS_90044A121_Black-Oxide Alloy Steel Socket Head Screw_10-32_2.5in:14
- Mate:233: ELEV_007_SUPBRK2:1 ↔ COTS_90044A121_Black-Oxide Alloy Steel Socket Head Screw_10-32_2.5in:15
- Mate:234: COTS_90044A121_Black-Oxide Alloy Steel Socket Head Screw_10-32_2.5in:13 ↔ ELEV_010_BOLTCOVER2:25
- Mate:235: ELEV_012_SUPBRK2_THRD:2 ↔ ELEV_010_BOLTCOVER2:25
- Mate:236: COTS_90044A121_Black-Oxide Alloy Steel Socket Head Screw_10-32_2.5in:16 ↔ ELEV_010_BOLTCOVER2:27
- Mate:237: COTS_90044A121_Black-Oxide Alloy Steel Socket Head Screw_10-32_2.5in:15 ↔ ELEV_010_BOLTCOVER2:28
- Mate:238: ELEV_010_BOLTCOVER2:26 ↔ COTS_90044A121_Black-Oxide Alloy Steel Socket Head Screw_10-32_2.5in:14
- Mate:239: ELEV_012_SUPBRK2_THRD:1 ↔ ELEV_010_BOLTCOVER2:26
- Mate:240: ELEV_012_SUPBRK2_THRD:1 ↔ ELEV_010_BOLTCOVER2:28
- Mate:241: ELEV_006_SUPBRK1_THRD:2 ↔ ELEV_010_BOLTCOVER2:37
- Mate:242: ELEV_006_SUPBRK1_THRD:2 ↔ ELEV_010_BOLTCOVER2:38
- Mate:243: ELEV_006_SUPBRK1_THRD:2 ↔ ELEV_010_BOLTCOVER2:38
- Mate:244: ELEV_006_SUPBRK1_THRD:2 ↔ ELEV_010_BOLTCOVER2:37
- Mate:245: COTS_90044A121_Black-Oxide Alloy Steel Socket Head Screw_10-32_2.5in:2 ↔ ELEV_010_BOLTCOVER2:40
- Mate:246: ELEV_010_BOLTCOVER2:39 ↔ COTS_90044A121_Black-Oxide Alloy Steel Socket Head Screw_10-32_2.5in:3
- Mate:247: ELEV_006_SUPBRK1_THRD:1 ↔ ELEV_010_BOLTCOVER2:39
- Mate:248: ELEV_006_SUPBRK1_THRD:1 ↔ ELEV_010_BOLTCOVER2:40
- Mate:249: COTS_91251A359_Black-Oxide Alloy Steel Socket Head Screw_10-32_2_3-4in:14 ↔ ELEV_010_BOLTCOVER2:49
- Mate:250: COTS_91251A359_Black-Oxide Alloy Steel Socket Head Screw_10-32_2_3-4in:13 ↔ ELEV_010_BOLTCOVER2:50
- Mate:251: COTS_91251A359_Black-Oxide Alloy Steel Socket Head Screw_10-32_2_3-4in:22 ↔ ELEV_010_BOLTCOVER2:51
- Mate:252: COTS_91251A359_Black-Oxide Alloy Steel Socket Head Screw_10-32_2_3-4in:16 ↔ ELEV_010_BOLTCOVER2:52
- Mate:253: COTS_90631A411_Low-Strength Steel Nylon-Insert Locknut_10-32:16 ↔ ELEV_010_BOLTCOVER2:52
- Mate:254: COTS_90631A411_Low-Strength Steel Nylon-Insert Locknut_10-32:22 ↔ ELEV_010_BOLTCOVER2:51
- Mate:255: COTS_90631A411_Low-Strength Steel Nylon-Insert Locknut_10-32:14 ↔ ELEV_010_BOLTCOVER2:49
- Mate:256: COTS_90631A411_Low-Strength Steel Nylon-Insert Locknut_10-32:15 ↔ ELEV_010_BOLTCOVER2:50
- Mate:257: ELEV_013_BAR5(12.000 in):1 ↔ WCP-0897_InlineBearingBlock:5
- Flush:29: ELEV_013_BAR5(12.000 in):1 ↔ WCP-0897_InlineBearingBlock:5
- Mate:258: ELEV_013_BAR5(12.000 in):1 ↔ WCP-0897_InlineBearingBlock:5
- Mate:259: ELEV_013_BAR5(12.000 in):1 ↔ WCP-0897_InlineBearingBlock:6
- Flush:30: ELEV_013_BAR5(12.000 in):1 ↔ WCP-0897_InlineBearingBlock:6
- Mate:260: ELEV_013_BAR5(12.000 in):1 ↔ WCP-0897_InlineBearingBlock:6
- Tangent:3: ELEV_003_BAR3(25.000 in):1 ↔ WCP-0897_InlineBearingBlock:5
- Tangent:4: ELEV_003_BAR3(25.000 in):1 ↔ WCP-0897_InlineBearingBlock:5
- Angle:5 (0 deg): ELEV_003_BAR3(25.000 in):1 ↔ ELEV_013_BAR5(12.000 in):1
- Angle:6 (0 deg): ELEV_003_BAR3(25.000 in):1 ↔ ELEV_013_BAR5(12.000 in):1
- Mate:261: ELEV_013_BAR5(12.000 in):2 ↔ WCP-0897_InlineBearingBlock:7
- Flush:31: ELEV_013_BAR5(12.000 in):2 ↔ WCP-0897_InlineBearingBlock:7
- Mate:262: ELEV_013_BAR5(12.000 in):2 ↔ WCP-0897_InlineBearingBlock:7
- Mate:263: ELEV_013_BAR5(12.000 in):2 ↔ WCP-0897_InlineBearingBlock:8
- Flush:32: ELEV_013_BAR5(12.000 in):2 ↔ WCP-0897_InlineBearingBlock:8
- Mate:264: ELEV_013_BAR5(12.000 in):2 ↔ WCP-0897_InlineBearingBlock:8
- Tangent:5: ELEV_003_BAR3(25.000 in):2 ↔ WCP-0897_InlineBearingBlock:7
- Angle:7 (0 deg): ELEV_004_BAR4(12.000 in):2 ↔ ELEV_013_BAR5(12.000 in):2
- Flush:33: ELEV_003_BAR3(25.000 in):2 ↔ ELEV_013_BAR5(12.000 in):2
- Flush:34: ELEV_013_BAR5(12.000 in):1 ↔ ELEV_013_BAR5(12.000 in):2
- Mate:265: ELEV_003_BAR3(25.000 in):1 ↔ ELEV_011_EXTRUENDCAP:8
- Mate:266: ELEV_003_BAR3(25.000 in):1 ↔ ELEV_011_EXTRUENDCAP:8
- Mate:267: ELEV_003_BAR3(25.000 in):1 ↔ ELEV_011_EXTRUENDCAP:8
- Mate:268: WCP-0897_InlineBearingBlock:8 ↔ COTS_91251A342_Black-Oxide Alloy Steel Socket Head Screw_.5in:9
- Mate:269: WCP-0897_InlineBearingBlock:8 ↔ COTS_91251A342_Black-Oxide Alloy Steel Socket Head Screw_.5in:9
- Mate:270: WCP-0897_InlineBearingBlock:5 ↔ COTS_91251A342_Black-Oxide Alloy Steel Socket Head Screw_.5in:10
- Mate:271: WCP-0897_InlineBearingBlock:5 ↔ COTS_91251A342_Black-Oxide Alloy Steel Socket Head Screw_.5in:10
- Mate:272: WCP-0897_InlineBearingBlock:7 ↔ COTS_91251A342_Black-Oxide Alloy Steel Socket Head Screw_.5in:8
- Mate:273: WCP-0897_InlineBearingBlock:7 ↔ COTS_91251A342_Black-Oxide Alloy Steel Socket Head Screw_.5in:8
- Mate:274: WCP-0897_InlineBearingBlock:6 ↔ COTS_91251A342_Black-Oxide Alloy Steel Socket Head Screw_.5in:7
- Mate:275: WCP-0897_InlineBearingBlock:6 ↔ COTS_91251A342_Black-Oxide Alloy Steel Socket Head Screw_.5in:7
- Mate:276: COTS_91251A342_Black-Oxide Alloy Steel Socket Head Screw_.5in:10 ↔ COTS_90633A411_Low-Strength Steel Thin Nylon-Insert Locknut_10-32:13
- Mate:277: ELEV_013_BAR5(12.000 in):1 ↔ COTS_90633A411_Low-Strength Steel Thin Nylon-Insert Locknut_10-32:13
- Mate:278: COTS_90633A411_Low-Strength Steel Thin Nylon-Insert Locknut_10-32:14 ↔ COTS_91251A342_Black-Oxide Alloy Steel Socket Head Screw_.5in:9
- Mate:279: ELEV_013_BAR5(12.000 in):2 ↔ COTS_90633A411_Low-Strength Steel Thin Nylon-Insert Locknut_10-32:14
- Mate:280: COTS_91251A342_Black-Oxide Alloy Steel Socket Head Screw_.5in:8 ↔ COTS_90633A411_Low-Strength Steel Thin Nylon-Insert Locknut_10-32:15
- Mate:281: ELEV_013_BAR5(12.000 in):2 ↔ COTS_90633A411_Low-Strength Steel Thin Nylon-Insert Locknut_10-32:15
- Mate:282: COTS_90633A411_Low-Strength Steel Thin Nylon-Insert Locknut_10-32:16 ↔ COTS_91251A342_Black-Oxide Alloy Steel Socket Head Screw_.5in:7
- Mate:283: ELEV_013_BAR5(12.000 in):1 ↔ COTS_90633A411_Low-Strength Steel Thin Nylon-Insert Locknut_10-32:16
- Mate:284: ELEV_001_BAR1(27.500 in):1 ↔ ELEV_015_CRSHBLCK1:1
- Mate:285: ELEV_001_BAR1(27.500 in):1 ↔ ELEV_015_CRSHBLCK1:1
- Mate:286: ELEV_001_BAR1(27.500 in):1 ↔ ELEV_015_CRSHBLCK1:1
- Mate:287: ELEV_001_BAR1(27.500 in):2 ↔ ELEV_015_CRSHBLCK1:2
- Mate:288: ELEV_001_BAR1(27.500 in):2 ↔ ELEV_015_CRSHBLCK1:2
- Mate:289: ELEV_001_BAR1(27.500 in):2 ↔ ELEV_015_CRSHBLCK1:2
- Mate:290: ELEV_001_BAR1(27.500 in):1 ↔ ELEV_016_SUPBAR1:1
- Mate:291: ELEV_001_BAR1(27.500 in):2 ↔ ELEV_016_SUPBAR1:1
- Mate:292: ELEV_001_BAR1(27.500 in):2 ↔ ELEV_016_SUPBAR1:1
- Mate:293: ELEV_001_BAR1(27.500 in):1 ↔ ELEV_016_SUPBAR1:2
- Mate:294: ELEV_001_BAR1(27.500 in):2 ↔ ELEV_016_SUPBAR1:2
- Mate:295: ELEV_001_BAR1(27.500 in):2 ↔ ELEV_016_SUPBAR1:2
- Mate:296: ELEV_016_SUPBAR1:2 ↔ COTS_90044A121_Black-Oxide Alloy Steel Socket Head Screw_10-32_2.5in:27
- Mate:297: ELEV_016_SUPBAR1:2 ↔ COTS_90044A121_Black-Oxide Alloy Steel Socket Head Screw_10-32_2.5in:27
- Mate:298: ELEV_016_SUPBAR1:2 ↔ COTS_90044A121_Black-Oxide Alloy Steel Socket Head Screw_10-32_2.5in:28
- Mate:299: ELEV_016_SUPBAR1:2 ↔ COTS_90044A121_Black-Oxide Alloy Steel Socket Head Screw_10-32_2.5in:28
- Mate:300: COTS_90044A121_Black-Oxide Alloy Steel Socket Head Screw_10-32_2.5in:28 ↔ COTS_90631A411_Low-Strength Steel Nylon-Insert Locknut_10-32:25
- Mate:301: ELEV_016_SUPBAR1:1 ↔ COTS_90631A411_Low-Strength Steel Nylon-Insert Locknut_10-32:25
- Mate:302: COTS_90044A121_Black-Oxide Alloy Steel Socket Head Screw_10-32_2.5in:27 ↔ COTS_90631A411_Low-Strength Steel Nylon-Insert Locknut_10-32:26
- Mate:303: ELEV_016_SUPBAR1:1 ↔ COTS_90631A411_Low-Strength Steel Nylon-Insert Locknut_10-32:26
- Mate:304: ELEV_016_SUPBAR1:2 ↔ ELEV_017_SPACER1:1
- Mate:305: ELEV_016_SUPBAR1:1 ↔ ELEV_017_SPACER1:1
- Mate:306: ELEV_016_SUPBAR1:2 ↔ ELEV_017_SPACER1:1
- Mate:307: ELEV_016_SUPBAR1:2 ↔ COTS_90044A121_Black-Oxide Alloy Steel Socket Head Screw_10-32_2.5in:29
- Mate:308: ELEV_016_SUPBAR1:2 ↔ COTS_90044A121_Black-Oxide Alloy Steel Socket Head Screw_10-32_2.5in:29
- Mate:309: COTS_90044A121_Black-Oxide Alloy Steel Socket Head Screw_10-32_2.5in:29 ↔ COTS_90631A411_Low-Strength Steel Nylon-Insert Locknut_10-32:27
- Mate:310: ELEV_016_SUPBAR1:1 ↔ COTS_90631A411_Low-Strength Steel Nylon-Insert Locknut_10-32:27
- Mate:312: ELEV_003_BAR3(25.000 in):1 ↔ ELEV_018_SUPBAR2:1
- Mate:313: ELEV_003_BAR3(25.000 in):1 ↔ ELEV_018_SUPBAR2:1
- Angle:8 (0 deg): ELEV_004_BAR4(12.000 in):1 ↔ ELEV_018_SUPBAR2:1
- Mate:314: ELEV_018_SUPBAR2:1 ↔ ELEV_018_SUPBAR2:2
- Mate:315: ELEV_018_SUPBAR2:1 ↔ ELEV_018_SUPBAR2:2
- Mate:316: ELEV_003_BAR3(25.000 in):1 ↔ ELEV_018_SUPBAR2:2
- Mate:317: ELEV_018_SUPBAR2:1 ↔ COTS_90044A121_Black-Oxide Alloy Steel Socket Head Screw_10-32_2.5in:31
- Mate:318: ELEV_018_SUPBAR2:1 ↔ COTS_90044A121_Black-Oxide Alloy Steel Socket Head Screw_10-32_2.5in:30
- Mate:319: ELEV_018_SUPBAR2:1 ↔ COTS_90044A121_Black-Oxide Alloy Steel Socket Head Screw_10-32_2.5in:30
- Mate:320: ELEV_018_SUPBAR2:1 ↔ COTS_90044A121_Black-Oxide Alloy Steel Socket Head Screw_10-32_2.5in:31
- Mate:321: COTS_90044A121_Black-Oxide Alloy Steel Socket Head Screw_10-32_2.5in:30 ↔ COTS_90631A411_Low-Strength Steel Nylon-Insert Locknut_10-32:29
- Mate:322: COTS_90044A121_Black-Oxide Alloy Steel Socket Head Screw_10-32_2.5in:31 ↔ COTS_90631A411_Low-Strength Steel Nylon-Insert Locknut_10-32:28
- Mate:323: ELEV_018_SUPBAR2:2 ↔ COTS_90631A411_Low-Strength Steel Nylon-Insert Locknut_10-32:28
- Mate:324: ELEV_018_SUPBAR2:2 ↔ COTS_90631A411_Low-Strength Steel Nylon-Insert Locknut_10-32:29
- Mate:325: ELEV_018_SUPBAR2:1 ↔ ELEV_017_SPACER1:2
- Mate:326: ELEV_018_SUPBAR2:1 ↔ ELEV_017_SPACER1:2
- Mate:327: ELEV_018_SUPBAR2:1 ↔ COTS_90044A121_Black-Oxide Alloy Steel Socket Head Screw_10-32_2.5in:32
- Mate:328: ELEV_018_SUPBAR2:1 ↔ COTS_90044A121_Black-Oxide Alloy Steel Socket Head Screw_10-32_2.5in:32
- Mate:329: COTS_90044A121_Black-Oxide Alloy Steel Socket Head Screw_10-32_2.5in:32 ↔ COTS_90631A411_Low-Strength Steel Nylon-Insert Locknut_10-32:30
- Mate:330: ELEV_018_SUPBAR2:2 ↔ COTS_90631A411_Low-Strength Steel Nylon-Insert Locknut_10-32:30
- Mate:331: COTS_90044A121_Black-Oxide Alloy Steel Socket Head Screw_10-32_2.5in:16 ↔ ELEV_010_BOLTCOVER2:61
- Mate:332: ELEV_012_SUPBRK2_THRD:2 ↔ ELEV_010_BOLTCOVER2:61
- Mate:333: ELEV_013_BAR5(12.000 in):1 ↔ ELEV_011_EXTRUENDCAP:9
- Mate:334: ELEV_013_BAR5(12.000 in):1 ↔ ELEV_011_EXTRUENDCAP:9
- Mate:335: ELEV_013_BAR5(12.000 in):1 ↔ ELEV_011_EXTRUENDCAP:9
- Mate:336: ELEV_013_BAR5(12.000 in):2 ↔ ELEV_011_EXTRUENDCAP:10
- Mate:337: ELEV_013_BAR5(12.000 in):2 ↔ ELEV_011_EXTRUENDCAP:10
- Mate:338: ELEV_013_BAR5(12.000 in):2 ↔ ELEV_011_EXTRUENDCAP:10
- Mate:339: ELEV_011_EXTRUENDCAP:3 ↔ ELEV_016_SUPBAR1:2
- Mate:340: ELEV_018_SUPBAR2:1 ↔ ELEV_011_EXTRUENDCAP:9
## Named parameters: sa_0 = 35585.8
note: some values were not read from the file. Shown as the stored number, unit unknown: "sa_0".
